# Autodesk Inventor assembly: benchtop-mesoSPIM-V2-1
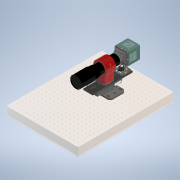
[picture p0: Inventor's stored thumbnail of the model, 180x180]
Saved by Autodesk Inventor 2021 (Build 250183000, 183)
## iProperties
Created: 2020-09-21
Part Number: benchtop-mesoSPIM-V2-1
Document SubType Name: Assembly
Designer: voigt
Author: voigt
## Documents named in this file (73)
- C:\Users\Public\mesoSPIM_design_benchtop\mesoSPIM\benchtop-mesoSPIM.iam
- C:\Users\Public\mesoSPIM_design_benchtop\library\Thorlabs\breadboards\PBG52522-Step.iam
- C:\Users\Public\mesoSPIM_design_benchtop\library\Thorlabs\accessoires\AV6_M.ipt
- C:\Users\Public\mesoSPIM_design_benchtop\library\Thorlabs\extrusions\XE25L375_M.ipt
- C:\Users\Public\mesoSPIM_design_benchtop\library\Thorlabs\extrusions\RM1S.ipt
- C:\Users\Public\mesoSPIM_design_benchtop\library\Thorlabs\extrusions\RM1G.ipt
- C:\Users\Public\mesoSPIM_design_benchtop\library\Thorlabs\extrusions\XE25L525_M.ipt
- C:\Users\Public\mesoSPIM_design_benchtop\library\Thorlabs\extrusions\XE25L350_M.ipt
- C:\Users\Public\mesoSPIM_design_benchtop\library\Thorlabs\accessoires\BBH1.ipt
- C:\Users\Public\mesoSPIM_design_benchtop\mesoSPIM\covers\Front_Cover_V1.ipt
- C:\Users\Public\mesoSPIM_design_benchtop\library\ASI\LS100_Vertical_Assembly.ipt
- C:\Users\Public\mesoSPIM_design_benchtop\library\ASI\ASI_mesoSPIM_Bridge.ipt
- C:\Users\Public\mesoSPIM_design_benchtop\library\ASI\LS-50HE ASSEMBLY (Centered Travel).ipt
- C:\Users\Public\mesoSPIM_design_benchtop\library\ASI\VTS-2112 DOVE RACK ASSEMBLY - (#DV6010 and #DV6020)_DV6010 ASSEMBLY with CDZ-SLIDE C.iam
- C:\Users\Public\mesoSPIM_design_benchtop\library\ASI\LS-50 LE ASSEMBLY_HOME.iam
- C:\Users\Public\mesoSPIM_design_benchtop\library\ASI\C60-3060-CMR-1011 - C-MOUNT TO LS50 SLIDE ADAPTER.ipt
- C:\Users\Public\mesoSPIM_design_benchtop\library\ASI\C60-3060-CMR - 3060 C-MOUNT ROTATING ASSEMBLY_C60-3060-CMR-Mo-ER20.iam
- C:\Users\Public\mesoSPIM_design_benchtop\library\ASI\LS-5012 - LS-BREADBOARD ADAPTER PLATE.ipt
- C:\Users\Public\mesoSPIM_design_benchtop\library\Thorlabs\rails\XT66SD.ipt
- C:\Users\Public\mesoSPIM_design_benchtop\library\Edmund_Optics\telecentric_objectives\62902_0_9x_F-Mount_PlatinumTL_Telecentric_lens.ipt
- C:\Users\Public\mesoSPIM_design_benchtop\library\Photometrics\Iris15_Volume_Correct.ipt
- C:\Users\Public\mesoSPIM_design_benchtop\library\Thorlabs\rails\XT66P2_M_single.ipt
- C:\Users\Public\mesoSPIM_design_benchtop\library\Thorlabs\posts\12_7_mm_posts\TR30.ipt
- C:\Users\Public\mesoSPIM_design_benchtop\library\Thorlabs\posts\post_mounts\PH20_M.ipt
- C:\Users\Public\mesoSPIM_design_benchtop\mesoSPIM\covers\Side_Cover_V1.ipt
- C:\Users\Public\mesoSPIM_design_benchtop\mesoSPIM\covers\Top_Cover_V1.ipt
- C:\Users\Public\mesoSPIM_design_benchtop\library\Thorlabs\extrusions\XE25H.ipt
- C:\Users\Public\mesoSPIM_design_benchtop\library\Thorlabs\posts\post_mounts\PH150_M.ipt
- C:\Users\Public\mesoSPIM_design_benchtop\library\Thorlabs\30mm_cage_system\cage_plates\CP33_M.ipt
- C:\Users\Public\mesoSPIM_design_benchtop\library\Thorlabs\posts\12_7_mm_posts\TR100M.ipt
- C:\Users\Public\mesoSPIM_design_benchtop\library\Thorlabs\30mm_cage_system\cage_rods\ER8_CageRod.ipt
- C:\Users\Public\mesoSPIM_design_benchtop\library\Thorlabs\optics\AC254-060-A-ML.ipt
- C:\Users\Public\mesoSPIM_design_benchtop\library\Thorlabs\accessoires\SM1FCA-APC-Fiberadapter.ipt
- C:\Users\Public\mesoSPIM_design_benchtop\library\Thorlabs\posts\post_mounts\PH40_M.ipt
- C:\Users\Public\mesoSPIM_design_benchtop\library\Thorlabs\posts\12_7_mm_posts\TR40M.ipt
- C:\Users\Public\mesoSPIM_design_benchtop\library\Thorlabs\30mm_cage_system\optics_mounts\KCB1E_M.ipt
- C:\Users\Public\mesoSPIM_design_benchtop\library\Thorlabs\optics\BBE1-E02-Step.ipt
- C:\Users\Public\mesoSPIM_design_benchtop\library\Thorlabs\optics\AC254-100-A-ML.ipt
- C:\Users\Public\mesoSPIM_design_benchtop\library\Optotune\EL-16-40\EL-16-40-TC-C (133-193-03-R0-01).iam
- C:\Users\Public\mesoSPIM_design_benchtop\library\Thorlabs\30mm_cage_system\SM1_tubes\SM1L10.ipt
- C:\Users\Public\mesoSPIM_design_benchtop\library\Thorlabs\accessoires\SM1A9.ipt
- C:\Users\Public\mesoSPIM_design_benchtop\library\Thorlabs\accessoires\SM1T2.ipt
- C:\Users\Public\mesoSPIM_design_benchtop\library\Thorlabs\accessoires\SM1NT.ipt
- C:\Users\Public\mesoSPIM_design_benchtop\library\Thorlabs\stages\XRN-B1_M-Micrometer-Baseplate.ipt
- C:\Users\Public\mesoSPIM_design_benchtop\library\Thorlabs\posts\post_mounts\PH75_M-Step.ipt
- C:\Users\Public\mesoSPIM_design_benchtop\library\Thorlabs\stages\XLN25P_M.ipt
- C:\Users\Public\mesoSPIM_design_benchtop\library\Thorlabs\stages\XRN25P_M.ipt
- C:\Users\Public\mesoSPIM_design_benchtop\library\Thorlabs\accessoires\AB90H.ipt
- C:\Users\Public\mesoSPIM_design_benchtop\library\Thorlabs\posts\12_7_mm_posts\TR75M.ipt
- C:\Users\Public\mesoSPIM_design_benchtop\library\Thorlabs\30mm_cage_system\cage_rods\ER0.5_CageRod.ipt
- C:\Users\Public\mesoSPIM_design_benchtop\library\Thorlabs\30mm_cage_system\cage_plates\CP30.ipt
- C:\Users\Public\mesoSPIM_design_benchtop\library\Thorlabs\30mm_cage_system\SM1_tubes\SM1L20.ipt
- C:\Users\Public\mesoSPIM_design_benchtop\library\Thorlabs\30mm_cage_system\SM1_tubes\SM1CPL.ipt
- C:\Users\Public\mesoSPIM_design_benchtop\library\Thorlabs\accessoires\BA1S_M.ipt
- C:\Users\Public\mesoSPIM_design_benchtop\library\Thorlabs\accessoires\MFF101_M_FlipMirror_SinglePart.ipt
- C:\Users\Public\mesoSPIM_design_benchtop\library\Thorlabs\optics\BB1-E02.ipt
- C:\Users\Public\mesoSPIM_design_benchtop\library\Thorlabs\60mm_cage_system\LCP03_M_modified_for_GVS411.ipt
- C:\Users\Public\mesoSPIM_design_benchtop\library\Thorlabs\galvos\GVS411-galvo-bracket-modified.ipt
- C:\Users\Public\mesoSPIM_design_benchtop\library\Thorlabs\galvos\GVS411_M.ipt
- C:\Users\Public\mesoSPIM_design_benchtop\mesoSPIM\excitation_path\components\60mm-blank-cageplate-LCP03M-Nikon-MOD.ipt
- C:\Users\Public\mesoSPIM_design_benchtop\library\Thorlabs\other\F-Mount-AdapterSM2NFM-Step.ipt
- C:\Users\Public\mesoSPIM_design_benchtop\library\Nikon\50mm_1_4G_body_disassembled.ipt
- C:\Users\Public\mesoSPIM_design_benchtop\library\Thorlabs\30mm_cage_system\cage_rods\ER4_CageRod.ipt
- C:\Users\Public\mesoSPIM_design_benchtop\mesoSPIM\sample_handling\Cuvette-Sampleholder\Cuvette-Sampleholder-with-base.iam
- C:\Users\Public\mesoSPIM_design_benchtop\library\Thorlabs\60mm_cage_system\LCFW5-wheel.ipt
- C:\Users\Public\mesoSPIM_design_benchtop\library\Robotis\MX-28T_R.ipt
- C:\Users\Public\mesoSPIM_design_benchtop\library\Robotis\FR07-S101.ipt
- C:\Users\nvladi\Documents\Inventor\mesoSPIM_design_benchtop_V2\library\Thorlabs\30mm_cage_system\cage_rods\ER_CageRod.ipt
- C:\Users\Public\mesoSPIM_design_benchtop\library\Lensation\T25M-12-155I.ipt
- C:\Users\Public\mesoSPIM_design_benchtop\mesoSPIM\detection_path\components\Lensagon1.2x-XT66P2M(ThorlabsRailCarriage).ipt
- C:\Users\Public\mesoSPIM_design_benchtop\library\Mouse_Brain\mousebrain2.ipt
- C:\Users\Public\mesoSPIM_design_benchtop\mesoSPIM\immersion_cuvette_mounts\ImmersionCuvetteAssembly.iam
- C:\Users\Public\mesoSPIM_design_benchtop\mesoSPIM\sample_handling\IDISCO-Sampleholder\Clamp-assembly.iam
## Components (172 placed, 71 different names)
1. AV6_M:4 — Mate:6, Mate:7
2. AV6_M:3 — Mate:8, Mate:9
3. AV6_M:2 — Mate:12, Mate:13
4. AV6_M:1 — Mate:10, Mate:11
5. PBG52522-Step:1 [sub-assembly] — Flush:1, Flush:2, Mate:5, Mate:6, Mate:7, Mate:8, Mate:9, Mate:10, Mate:11, Mate:12, Mate:13, Mate:14, Mate:15, Angle:1, Mate:16, Mate:17, Angle:2, Mate:18, Mate:19, Angle:3, Mate:20, Mate:21, Angle:4, Mate:32, Mate:48, Mate:49, Mate:50, Angle:5, Mate:51, Angle:6, Mate:72, Mate:107, Angle:15, Mate:109, Mate:110, Angle:16, Flush:45, Mate:139, Mate:140, Angle:18, Mate:141, Mate:142, Angle:19, Flush:49, Angle:20, Mate:191, Mate:192, Angle:23, Angle:24, Mate:196, Mate:197, Mate:198, Angle:25, Mate:199, Mate:200, Angle:26, Mate:238, Mate:239, Angle:28, Angle:30, Mate:243, Mate:324, Tangent:1, Mate:325, Mate:331, Angle:44, Mate:382, Angle:46, Tangent:2, Mate:385, Angle:47
6. LS100_Vertical_Assembly:1 — Mate:48, Mate:50, Angle:5, Mate:52, Mate:53
7. LS100_Vertical_Assembly:2 — Mate:49, Mate:51, Angle:6, Mate:54
8. ASI_mesoSPIM_Bridge:1 — Mate:52, Mate:53, Mate:54, Mate:55, Flush:36
9. LS-50HE ASSEMBLY (Centered Travel):1 — Mate:55, Flush:36, Mate:56, Mate:57, Angle:7, Mate:58, Mate:59, Angle:8
10. VTS-2112 DOVE RACK ASSEMBLY - (#DV6010 and #DV6020)_DV6010 ASSEMBLY with CDZ-SLIDE C:1 [sub-assembly] — Mate:57, Angle:7, Mate:58, Mate:59, Mate:60, Mate:61, Mate:62
11. LS-50 LE ASSEMBLY_HOME:1 [sub-assembly] — Mate:60, Mate:61, Mate:62, Angle:8, Mate:63, Mate:64, Mate:65
12. C60-3060-CMR-1011 - C-MOUNT TO LS50 SLIDE ADAPTER:1 — Mate:63, Mate:64, Mate:65, Mate:66, Mate:67
13. C60-3060-CMR - 3060 C-MOUNT ROTATING ASSEMBLY_C60-3060-CMR-Mo-ER20:1 [sub-assembly] — Mate:66, Mate:67, Mate:367, VerticalPos
14. LS-5012 - LS-BREADBOARD ADAPTER PLATE:1 — Mate:70, Angle:9, Mate:72, Mate:77
15. LS-50 LE ASSEMBLY_HOME:2 [sub-assembly] — Mate:70, Angle:9, Mate:73, Mate:74, Angle:10, Mate:77
16. XT66SD:1 — Mate:73, Mate:74, Angle:10, Mate:75, Mate:76, Angle:11, Mate:82, Mate:83, Mate:84, Mate:85
17. 62902_0_9x_F-Mount_PlatinumTL_Telecentric_lens:1 — Mate:78, Mate:81
18. Lensagon-T25M-12-155I:1 — Insert:3, Insert:7
19. Lensagon1.2x-XT66P2M(ThorlabsRailCarriage):1 — Mate:384, Flush:72, Flush:73, Insert:7
20. Iris15_Volume_Correct:1 — Angle:11, Mate:81, Insert:3, Insert:8
21. XT66P2_M_single:1 — Mate:82, Mate:83, Mate:96, Mate:97
22. XT66P2_M_single:2 — Mate:84, Mate:85, Mate:384, Flush:72, Flush:73
23. TR30:1 — Insert:8
24. PH20_M:1 — Mate:96, Mate:97
25. KCB1E_M:2 — Mate:184, Mate:185, Mate:186, Mate:187, Mate:188, Mate:190, Angle:21, Angle:36
26. BBE1-E02-Step:2 — Mate:189, Mate:190, Angle:21
27. CP33_M:2 — Mate:117, Mate:118, Mate:122
28. TR100M:1 — Mate:119
29. TR100M:2 — Mate:121, Mate:122
30. CP33_M:3 — Mate:124, Mate:129, Mate:131, Mate:133
31. CP33_M:4 — Mate:123, Flush:48, Mate:294
32. ER8_CageRod:1 — Mate:186, Mate:308
33. ER8_CageRod:2 — Mate:188, Mate:307
34. ER8_CageRod:3 — Mate:129, Mate:187, Mate:294
35. AC254-060-A-ML:1 — Mate:130, Mate:131
36. SM1FCA-APC-Fiberadapter:1 — Mate:132, Flush:48, Mate:133
37. PH150_M:1 — Mate:109, Mate:110, Angle:16, Mate:118, Mate:121
38. PH150_M:2 — Mate:107, Angle:15, Mate:119
39. LCP03_M_modified_for_GVS411:1 — Mate:337, Mate:338, Angle:39, Mate:349, Insert:2
40. GVS411-galvo-bracket-modified:1 — Mate:337, Mate:338, Mate:339, Angle:38, Angle:39, Mate:341
41. GVS411_M:1 — Mate:339, Angle:38, Mate:340, Mate:341, Mate:348
42. 60mm-blank-cageplate-LCP03M-Nikon-MOD:1 — Mate:344, Mate:345, Mate:347, Flush:66, Mate:350, Flush:67, Insert:1
43. F-Mount-AdapterSM2NFM-Step:1 — Mate:344, Mate:345, Mate:346
44. 50mm_1_4G_body_disassembled:1 — Mate:346, Mate:347, Mate:348
45. TR75M:2 — Mate:272
46. AB90H:1 — Mate:264, Mate:265, Flush:62
47. KCB1E_M:4 — Mate:254, Mate:255, Mate:258, Mate:259, Mate:265, Flush:62
48. BBE1-E02-Step:5 — Mate:258, Mate:259
49. XLN25P_M:1 — Mate:244, Mate:245, Mate:248, Mate:264
50. PH75_M-Step:2 — Mate:192, Angle:23, Mate:272
51. XRN-B1_M-Micrometer-Baseplate:1 — Mate:191, Angle:24, Mate:196, Mate:244, Mate:245
52. EL-16-40-TC-C (133-193-03-R0-01):1 [sub-assembly] — Mate:174, Mate:175, Mate:178, Mate:179
53. SM1L10:2 — Mate:176, Mate:177, Mate:181, Mate:182, Mate:183, Mate:185
54. SM1A9:1 — Mate:178, Mate:179, Mate:180
55. SM1T2:1 — Mate:180, Mate:181
56. SM1NT:1 — Mate:182, Mate:183
57. PH40_M:1 — Mate:139, Mate:140, Angle:18, Mate:148
58. PH40_M:2 — Mate:141, Mate:142, Angle:19, Mate:150
59. CP33_M:5 — Mate:147, Mate:148, Mate:153, Mate:154, Mate:155, Mate:156, Flush:53, Mate:159, Mate:160
60. CP33_M:6 — Mate:149, Mate:150, Mate:161, Mate:162
61. CP33_M:7 — Mate:151, Mate:157, Flush:54, Mate:169
62. ER8_CageRod:4 — Mate:156, Flush:51
63. ER8_CageRod:5 — Mate:155, Flush:50, Flush:51, Flush:52, Mate:157
64. ER8_CageRod:6 — Mate:154, Flush:52
65. ER8_CageRod:7 — Mate:153, Flush:50, Flush:53, Flush:54, Mate:164, Mate:165
66. TR40M:1 — Mate:159, Mate:160
67. TR40M:2 — Mate:161, Mate:162
68. KCB1E_M:1 — Mate:163, Mate:164, Mate:165, Mate:167, Mate:173, Mate:175, Mate:177
69. BBE1-E02-Step:1 — Mate:166, Mate:167, Angle:20
70. AC254-100-A-ML:1 — Mate:168, Mate:169
71. AC254-100-A-ML:2
72. ER4_CageRod:12 — Mate:349, Flush:66
73. ER4_CageRod:19 — Insert:1
74. ER4_CageRod:20 — Insert:2
75. ER4_CageRod:13 — Mate:350, Flush:67
76. LCP03_M_modified_for_GVS411:2 — Mate:352, Mate:353, Angle:41, Angle:43, Insert:10, Insert:11
77. GVS411-galvo-bracket-modified:2 — Mate:352, Mate:353, Angle:41, Mate:354, Angle:42, Mate:356
78. GVS411_M:2 — Mate:354, Angle:42, Mate:355, Mate:356, Mate:362
79. 60mm-blank-cageplate-LCP03M-Nikon-MOD:2 — Angle:43, Mate:358, Mate:359, Mate:361, Mate:365, Flush:70, Flush:71, Mate:366
80. F-Mount-AdapterSM2NFM-Step:2 — Mate:358, Mate:359, Mate:360
81. 50mm_1_4G_body_disassembled:2 — Mate:360, Mate:361, Mate:362
82. ER4_CageRod:14 — Mate:365, Flush:70
83. ER4_CageRod:16 — Flush:71, Mate:366
84. TR75M:4 — Mate:278
85. AB90H:2 — Mate:266, Mate:267, Flush:63
86. KCB1E_M:5 — Mate:256, Mate:257, Mate:261, Mate:267, Flush:63
87. BBE1-E02-Step:4 — Mate:260, Mate:261
88. XRN25P_M:1 — Mate:246, Mate:247, Mate:249, Mate:266
89. PH40_M:3 — Mate:197, Mate:198, Angle:25, Mate:205
90. PH40_M:4 — Mate:199, Mate:200, Angle:26, Mate:206
91. CP33_M:9 — Mate:201, Mate:205, Mate:207, Mate:208, Mate:211, Mate:212, Mate:213, Mate:214
92. CP33_M:10 — Mate:202, Mate:206, Mate:209, Mate:210, Flush:58
93. TR40M:3 — Mate:207, Mate:208
94. TR40M:4 — Mate:209, Mate:210
95. ER8_CageRod:8 — Mate:211, Flush:57, Flush:59
96. ER8_CageRod:9 — Mate:213, Flush:56, Flush:58, Mate:216, Mate:217, Mate:222
97. ER8_CageRod:10 — Mate:214, Flush:55, Flush:56, Flush:57
98. ER8_CageRod:11 — Mate:212, Flush:55
99. ER4_CageRod:21 — Insert:11
100. ER4_CageRod:22 — Insert:10
101. KCB1E_M:3 — Mate:215, Mate:216, Mate:217, Mate:219, Angle:27, Mate:227, Mate:228, Mate:229, Mate:231
102. BBE1-E02-Step:3 — Mate:218, Mate:219, Angle:27
103. CP33_M:11 — Mate:220, Flush:59, Mate:224
104. CP33_M:12 — Mate:221, Mate:222, Mate:226
105. AC254-100-A-ML:3 — Mate:223, Mate:224
106. AC254-100-A-ML:4 — Mate:225, Mate:226, Mate:227
107. SM1L10:3 — Mate:228, Mate:229, Mate:230, Mate:236, Mate:237, Mate:292
108. EL-16-40-TC-C (133-193-03-R0-01):2 [sub-assembly] — Mate:230, Mate:231, Mate:232, Mate:233
109. SM1A9:3 — Mate:232, Mate:233, Mate:234, Mate:235
110. SM1T2:2 — Mate:234, Mate:235
111. SM1NT:2 — Mate:236, Mate:237
112. XRN-B1_M-Micrometer-Baseplate:2 — Mate:238, Angle:30, Mate:243, Mate:246, Mate:247
113. PH75_M-Step:3 — Mate:239, Angle:28, Mate:278
114. CP33_M:13 — Mate:299, Mate:301, Mate:303, Mate:305, Mate:317
115. KCB1E_M:6 — Mate:292, Mate:296, Angle:32, Angle:35, Mate:300, Mate:302, Mate:314
116. KCB1E_M:7 — Mate:297, Angle:33, Angle:34, Mate:298, Angle:35, Mate:304, Mate:306, Mate:311, Mate:312, Mate:313, Mate:317, Mate:319, Mate:320
117. BBE1-E02-Step:6 — Mate:295, Mate:296, Angle:32
118. BBE1-E02-Step:7 — Mate:297, Angle:33, Angle:34, Mate:298
119. ER0.5_CageRod:1 — Mate:299, Mate:300, Mate:314
120. ER0.5_CageRod:2 — Mate:301, Mate:302
121. ER0.5_CageRod:3 — Mate:303, Mate:304, Mate:313
122. ER0.5_CageRod:4 — Mate:305, Mate:306
123. CP30:1 — Mate:307, Mate:308, Mate:309, Mate:310
124. SM1L20:1 — Mate:309, Mate:310, Mate:316
125. SM1L20:2 — Mate:311, Mate:312, Mate:316, Mate:318
126. SM1CPL:1 — Mate:318
127. TR100M:3 — Mate:319, Mate:320, Mate:321
128. PH150_M:3 — Mate:321, Mate:322, Mate:323
129. BA1S_M:1 — Mate:322, Mate:323, Mate:324, Tangent:1
130. BA1S_M:2 — Mate:325, Mate:326, Mate:327
131. PH75_M-Step:6 — Mate:326, Mate:327, Mate:328
132. TR75M:5 — Mate:328, Mate:329, Mate:330
133. MFF101_M_FlipMirror_SinglePart:1 — Mate:329, Mate:330, Angle:36, Mate:331, Mate:332, Mate:333
134. BB1-E02:1 — Mate:332, Mate:333
135. mousebrain2:1
136. TR40M:5 — Mate:367, VerticalPos, Mate:369, Mate:370, Insert:9
137. Clamp-assembly:1 [sub-assembly] — Insert:9, Angle:47
138. Cuvette-Sampleholder-with-base:1 [sub-assembly] — Mate:369, Mate:370, Angle:44
139. LCFW5-wheel:1 — Mate:371, Mate:372, Mate:373, Mate:383
140. MX-28T_R:1 — Mate:373, Mate:374, Mate:375, Mate:376, Mate:383
141. FR07-S101:1 — Mate:374, Mate:375, Mate:376, Mate:377, Mate:378
142. TR30:2 — Mate:377, Mate:378, Mate:379
143. PH20_M:2 — Mate:379, Mate:381, Angle:45
144. BA1S_M:3 — Mate:381, Mate:382, Angle:45, Angle:46, Tangent:2
145. ImmersionCuvetteAssembly:1 [sub-assembly] — Mate:385
146. XE25H:1 — Mate:103, Angle:14, Mate:104, Flush:43
147. XE25H:2 — Mate:105, Mate:106, Flush:44
148. XE25L525_M:1 — Mate:29, Flush:17, Flush:18, Mate:101, Flush:40, Flush:42
149. XE25L525_M:2 — Mate:28, Flush:15, Flush:16, Mate:100, Flush:38
150. XE25L375_M:5 — Mate:27, Flush:13, Flush:14, Flush:19, Mate:30, Flush:20, Mate:103, Flush:43, Mate:105, Flush:44
151. XE25L375_M:6 — Mate:26, Flush:11, Flush:12, Flush:41
152. RM1G:1 — Mate:22, Flush:3, Flush:4, Mate:28, Flush:15, Flush:16
153. RM1G:2 — Mate:24, Flush:7, Flush:8, Mate:26, Flush:11, Flush:12, Mate:29, Flush:17, Flush:18
154. RM1G:3 — Mate:25, Flush:9, Flush:10, Mate:27, Flush:13, Flush:14, Mate:104
155. RM1G:4 — Mate:23, Flush:5, Flush:6, Mate:102, Mate:106
156. XE25L375_M:1 — Mate:14, Mate:15, Angle:1, Mate:22, Flush:3, Flush:4, Flush:37
157. XE25L375_M:2 — Mate:16, Mate:17, Angle:2, Mate:24, Flush:7, Flush:8, Flush:39
158. XE25L375_M:3 — Mate:18, Mate:19, Angle:3, Mate:25, Flush:9, Flush:10
159. XE25L375_M:4 — Mate:20, Mate:21, Angle:4, Mate:23, Flush:5, Flush:6, Flush:21, Mate:31
160. Front_Cover_V1:1 — Mate:41, Mate:42, Mate:43
161. BBH1:1 — Mate:39, Flush:35, Mate:40
162. RM1S:1 — Mate:33, Flush:22, Flush:23
163. RM1S:2 — Mate:34, Flush:24, Flush:25, Flush:33, Flush:34, Mate:38
164. RM1S:3 — Flush:28, Mate:36, Flush:29, Flush:30, Mate:37, Flush:31, Flush:32
165. RM1S:4 — Mate:35, Flush:26, Flush:27
166. XE25L375_M:7 — Flush:19, Mate:30, Flush:20, Mate:34, Flush:24, Flush:25, Flush:28, Mate:36, Flush:29, Flush:30, Mate:43, Angle:14
167. XE25L375_M:8 — Flush:21, Mate:31, Mate:32, Mate:33, Flush:22, Flush:23, Mate:35, Flush:26, Flush:27, Mate:39, Flush:35
168. XE25L350_M:1 — Mate:37, Flush:31, Flush:32, Mate:41, Mate:42
169. XE25L350_M:2 — Flush:33, Flush:34, Mate:38
170. Side_Cover_V1:1 — Mate:100, Flush:37, Flush:38
171. Side_Cover_V1:2 — Mate:101, Flush:39, Flush:40
172. Top_Cover_V1:1 — Mate:102, Flush:41, Flush:42
## Relationships (418: Mate 302, Flush 67, Angle 39, Insert 8, Tangent 2)
- Flush:1 (135 mm): PBG52522-Step:1
- Flush:2 (225 mm): PBG52522-Step:1
- Mate:5 (-100 mm): PBG52522-Step:1
- Mate:6: AV6_M:4 ↔ PBG52522-Step:1
- Mate:7: AV6_M:4 ↔ PBG52522-Step:1
- Mate:8: AV6_M:3 ↔ PBG52522-Step:1
- Mate:9: AV6_M:3 ↔ PBG52522-Step:1
- Mate:10: AV6_M:1 ↔ PBG52522-Step:1
- Mate:11: AV6_M:1 ↔ PBG52522-Step:1
- Mate:12: AV6_M:2 ↔ PBG52522-Step:1
- Mate:13: AV6_M:2 ↔ PBG52522-Step:1
- Mate:14: PBG52522-Step:1 ↔ XE25L375_M:1
- Mate:15: PBG52522-Step:1 ↔ XE25L375_M:1
- Angle:1 (0 deg): PBG52522-Step:1 ↔ XE25L375_M:1
- Mate:16: PBG52522-Step:1 ↔ XE25L375_M:2
- Mate:17: PBG52522-Step:1 ↔ XE25L375_M:2
- Angle:2 (0 deg): PBG52522-Step:1 ↔ XE25L375_M:2
- Mate:18: PBG52522-Step:1 ↔ XE25L375_M:3
- Mate:19: PBG52522-Step:1 ↔ XE25L375_M:3
- Angle:3 (0 deg): PBG52522-Step:1 ↔ XE25L375_M:3
- Mate:20: PBG52522-Step:1 ↔ XE25L375_M:4
- Mate:21: PBG52522-Step:1 ↔ XE25L375_M:4
- Angle:4 (0 deg): PBG52522-Step:1 ↔ XE25L375_M:4
- Mate:22: RM1G:1 ↔ XE25L375_M:1
- Flush:3: RM1G:1 ↔ XE25L375_M:1
- Flush:4: RM1G:1 ↔ XE25L375_M:1
- Mate:23: RM1G:4 ↔ XE25L375_M:4
- Flush:5: RM1G:4 ↔ XE25L375_M:4
- Flush:6: RM1G:4 ↔ XE25L375_M:4
- Mate:24: RM1G:2 ↔ XE25L375_M:2
- Flush:7: RM1G:2 ↔ XE25L375_M:2
- Flush:8: RM1G:2 ↔ XE25L375_M:2
- Mate:25: RM1G:3 ↔ XE25L375_M:3
- Flush:9: RM1G:3 ↔ XE25L375_M:3
- Flush:10: RM1G:3 ↔ XE25L375_M:3
- Mate:26: XE25L375_M:6 ↔ RM1G:2
- Flush:11: XE25L375_M:6 ↔ RM1G:2
- Flush:12: XE25L375_M:6 ↔ RM1G:2
- Mate:27: XE25L375_M:5 ↔ RM1G:3
- Flush:13: XE25L375_M:5 ↔ RM1G:3
- Flush:14: XE25L375_M:5 ↔ RM1G:3
- Mate:28: XE25L525_M:2 ↔ RM1G:1
- Flush:15: XE25L525_M:2 ↔ RM1G:1
- Flush:16: XE25L525_M:2 ↔ RM1G:1
- Mate:29: XE25L525_M:1 ↔ RM1G:2
- Flush:17: XE25L525_M:1 ↔ RM1G:2
- Flush:18: XE25L525_M:1 ↔ RM1G:2
- Flush:19: XE25L375_M:5 ↔ XE25L375_M:7
- Mate:30: XE25L375_M:5 ↔ XE25L375_M:7
- Flush:20: XE25L375_M:5 ↔ XE25L375_M:7
- Flush:21 (-25 mm): XE25L375_M:4 ↔ XE25L375_M:8
- Mate:31: XE25L375_M:4 ↔ XE25L375_M:8
- Mate:32: PBG52522-Step:1 ↔ XE25L375_M:8
- Mate:33: RM1S:1 ↔ XE25L375_M:8
- Flush:22: RM1S:1 ↔ XE25L375_M:8
- Flush:23: RM1S:1 ↔ XE25L375_M:8
- Mate:34: RM1S:2 ↔ XE25L375_M:7
- Flush:24: RM1S:2 ↔ XE25L375_M:7
- Flush:25: RM1S:2 ↔ XE25L375_M:7
- Mate:35: RM1S:4 ↔ XE25L375_M:8
- Flush:26: RM1S:4 ↔ XE25L375_M:8
- Flush:27: RM1S:4 ↔ XE25L375_M:8
- Flush:28: RM1S:3 ↔ XE25L375_M:7
- Mate:36: RM1S:3 ↔ XE25L375_M:7
- Flush:29: RM1S:3 ↔ XE25L375_M:7
- Flush:30: RM1S:3 ↔ XE25L375_M:7
- Mate:37: RM1S:3 ↔ XE25L350_M:1
- Flush:31: RM1S:3 ↔ XE25L350_M:1
- Flush:32: RM1S:3 ↔ XE25L350_M:1
- Flush:33: RM1S:2 ↔ XE25L350_M:2
- Flush:34: RM1S:2 ↔ XE25L350_M:2
- Mate:38: RM1S:2 ↔ XE25L350_M:2
- Mate:39: BBH1:1 ↔ XE25L375_M:8
- Flush:35: BBH1:1 ↔ XE25L375_M:8
- Mate:40 (62.5 mm): BBH1:1
- Mate:41: Front_Cover_V1:1 ↔ XE25L350_M:1
- Mate:42 (-6 mm): Front_Cover_V1:1 ↔ XE25L350_M:1
- Mate:43 (-2 mm): Front_Cover_V1:1 ↔ XE25L375_M:7
- Mate:44
- Mate:45
- Mate:48: PBG52522-Step:1 ↔ LS100_Vertical_Assembly:1
- Mate:49: PBG52522-Step:1 ↔ LS100_Vertical_Assembly:2
- Mate:50: PBG52522-Step:1 ↔ LS100_Vertical_Assembly:1
- Angle:5 (0 deg): PBG52522-Step:1 ↔ LS100_Vertical_Assembly:1
- Mate:51: PBG52522-Step:1 ↔ LS100_Vertical_Assembly:2
- Angle:6 (0 deg): PBG52522-Step:1 ↔ LS100_Vertical_Assembly:2
- Mate:52: LS100_Vertical_Assembly:1 ↔ ASI_mesoSPIM_Bridge:1
- Mate:53: LS100_Vertical_Assembly:1 ↔ ASI_mesoSPIM_Bridge:1
- Mate:54: LS100_Vertical_Assembly:2 ↔ ASI_mesoSPIM_Bridge:1
- Mate:55: ASI_mesoSPIM_Bridge:1 ↔ LS-50HE ASSEMBLY (Centered Travel):1
- Flush:36: ASI_mesoSPIM_Bridge:1 ↔ LS-50HE ASSEMBLY (Centered Travel):1
- Mate:56 (12.5 mm): LS-50HE ASSEMBLY (Centered Travel):1
- Mate:57: LS-50HE ASSEMBLY (Centered Travel):1 ↔ VTS-2112 DOVE RACK ASSEMBLY - (#DV6010 and #DV6020)_DV6010 ASSEMBLY with CDZ-SLIDE C:1
- Angle:7 (0 deg): LS-50HE ASSEMBLY (Centered Travel):1 ↔ VTS-2112 DOVE RACK ASSEMBLY - (#DV6010 and #DV6020)_DV6010 ASSEMBLY with CDZ-SLIDE C:1
- Mate:58: LS-50HE ASSEMBLY (Centered Travel):1 ↔ VTS-2112 DOVE RACK ASSEMBLY - (#DV6010 and #DV6020)_DV6010 ASSEMBLY with CDZ-SLIDE C:1
- Mate:59: LS-50HE ASSEMBLY (Centered Travel):1 ↔ VTS-2112 DOVE RACK ASSEMBLY - (#DV6010 and #DV6020)_DV6010 ASSEMBLY with CDZ-SLIDE C:1
- Mate:60: VTS-2112 DOVE RACK ASSEMBLY - (#DV6010 and #DV6020)_DV6010 ASSEMBLY with CDZ-SLIDE C:1 ↔ LS-50 LE ASSEMBLY_HOME:1
- Mate:61: VTS-2112 DOVE RACK ASSEMBLY - (#DV6010 and #DV6020)_DV6010 ASSEMBLY with CDZ-SLIDE C:1 ↔ LS-50 LE ASSEMBLY_HOME:1
- Mate:62: VTS-2112 DOVE RACK ASSEMBLY - (#DV6010 and #DV6020)_DV6010 ASSEMBLY with CDZ-SLIDE C:1 ↔ LS-50 LE ASSEMBLY_HOME:1
- Angle:8 (0 deg): LS-50HE ASSEMBLY (Centered Travel):1 ↔ LS-50 LE ASSEMBLY_HOME:1
- Mate:63: LS-50 LE ASSEMBLY_HOME:1 ↔ C60-3060-CMR-1011 - C-MOUNT TO LS50 SLIDE ADAPTER:1
- Mate:64: LS-50 LE ASSEMBLY_HOME:1 ↔ C60-3060-CMR-1011 - C-MOUNT TO LS50 SLIDE ADAPTER:1
- Mate:65: LS-50 LE ASSEMBLY_HOME:1 ↔ C60-3060-CMR-1011 - C-MOUNT TO LS50 SLIDE ADAPTER:1
- Mate:66: C60-3060-CMR-1011 - C-MOUNT TO LS50 SLIDE ADAPTER:1 ↔ C60-3060-CMR - 3060 C-MOUNT ROTATING ASSEMBLY_C60-3060-CMR-Mo-ER20:1
- Mate:67: C60-3060-CMR-1011 - C-MOUNT TO LS50 SLIDE ADAPTER:1 ↔ C60-3060-CMR - 3060 C-MOUNT ROTATING ASSEMBLY_C60-3060-CMR-Mo-ER20:1
- Mate:70: LS-5012 - LS-BREADBOARD ADAPTER PLATE:1 ↔ LS-50 LE ASSEMBLY_HOME:2
- Angle:9 (0 deg): LS-5012 - LS-BREADBOARD ADAPTER PLATE:1 ↔ LS-50 LE ASSEMBLY_HOME:2
- Mate:72: PBG52522-Step:1 ↔ LS-5012 - LS-BREADBOARD ADAPTER PLATE:1
- Mate:73: LS-50 LE ASSEMBLY_HOME:2 ↔ XT66SD:1
- Mate:74: LS-50 LE ASSEMBLY_HOME:2 ↔ XT66SD:1
- Angle:10 (0 deg): LS-50 LE ASSEMBLY_HOME:2 ↔ XT66SD:1
- Mate:75: XT66SD:1
- Mate:76: XT66SD:1
- Mate:77: LS-5012 - LS-BREADBOARD ADAPTER PLATE:1 ↔ LS-50 LE ASSEMBLY_HOME:2
- Mate:78: 62902_0_9x_F-Mount_PlatinumTL_Telecentric_lens:1
- Angle:11 (0 deg): XT66SD:1 ↔ Iris15_Volume_Correct:1
- Mate:81: 62902_0_9x_F-Mount_PlatinumTL_Telecentric_lens:1 ↔ Iris15_Volume_Correct:1
- Mate:82: XT66SD:1 ↔ XT66P2_M_single:1
- Mate:83: XT66SD:1 ↔ XT66P2_M_single:1
- Mate:84: XT66SD:1 ↔ XT66P2_M_single:2
- Mate:85: XT66SD:1 ↔ XT66P2_M_single:2
- Mate:96: XT66P2_M_single:1 ↔ PH20_M:1
- Mate:97: XT66P2_M_single:1 ↔ PH20_M:1
- Mate:100: XE25L525_M:2 ↔ Side_Cover_V1:1
- Flush:37: XE25L375_M:1 ↔ Side_Cover_V1:1
- Flush:38: XE25L525_M:2 ↔ Side_Cover_V1:1
- Mate:101: XE25L525_M:1 ↔ Side_Cover_V1:2
- Flush:39: XE25L375_M:2 ↔ Side_Cover_V1:2
- Flush:40: XE25L525_M:1 ↔ Side_Cover_V1:2
- Mate:102: RM1G:4 ↔ Top_Cover_V1:1
- Flush:41: XE25L375_M:6 ↔ Top_Cover_V1:1
- Flush:42: XE25L525_M:1 ↔ Top_Cover_V1:1
- Mate:103: XE25H:1 ↔ XE25L375_M:5
- Angle:14 (0 deg): XE25H:1 ↔ XE25L375_M:7
- Mate:104: XE25H:1 ↔ RM1G:3
- Flush:43 (5.75 mm): XE25H:1 ↔ XE25L375_M:5
- Mate:105: XE25H:2 ↔ XE25L375_M:5
- Mate:106: XE25H:2 ↔ RM1G:4
- Flush:44 (5.75 mm): XE25H:2 ↔ XE25L375_M:5
- Mate:107: PBG52522-Step:1 ↔ PH150_M:2
- Angle:15 (0 deg): PBG52522-Step:1 ↔ PH150_M:2
- Mate:109: PBG52522-Step:1 ↔ PH150_M:1
- Mate:110: PBG52522-Step:1 ↔ PH150_M:1
- Angle:16 (0 deg): PBG52522-Step:1 ↔ PH150_M:1
- Flush:45 (215 mm): PBG52522-Step:1
- Flush:46 (-100 mm)
- Flush:47 (100 mm)
- Mate:111
- Mate:112
- Mate:113
- Mate:114
- Mate:117: CP33_M:2
- Mate:118: CP33_M:2 ↔ PH150_M:1
- Mate:119: TR100M:1 ↔ PH150_M:2
- Mate:121: TR100M:2 ↔ PH150_M:1
- Mate:122: CP33_M:2 ↔ TR100M:2
- Mate:123: CP33_M:4
- Mate:124: CP33_M:3
- Mate:129: CP33_M:3 ↔ ER8_CageRod:3
- Mate:130: AC254-060-A-ML:1
- Mate:131: CP33_M:3 ↔ AC254-060-A-ML:1
- Mate:132: SM1FCA-APC-Fiberadapter:1
- Flush:48 (-0.5 mm): CP33_M:4 ↔ SM1FCA-APC-Fiberadapter:1
- Mate:133 (50 mm): CP33_M:3 ↔ SM1FCA-APC-Fiberadapter:1
- Mate:139: PBG52522-Step:1 ↔ PH40_M:1
- Mate:140: PBG52522-Step:1 ↔ PH40_M:1
- Angle:18 (0 deg): PBG52522-Step:1 ↔ PH40_M:1
- Mate:141: PBG52522-Step:1 ↔ PH40_M:2
- Mate:142: PBG52522-Step:1 ↔ PH40_M:2
- Angle:19 (0 deg): PBG52522-Step:1 ↔ PH40_M:2
- Flush:49 (70 mm): PBG52522-Step:1
- Mate:143
- Mate:144
- Mate:145
- Mate:146
- Mate:147: CP33_M:5
- Mate:148: PH40_M:1 ↔ CP33_M:5
- Mate:149: CP33_M:6
- Mate:150: PH40_M:2 ↔ CP33_M:6
- Mate:151: CP33_M:7
- Mate:153: CP33_M:5 ↔ ER8_CageRod:7
- Mate:154: CP33_M:5 ↔ ER8_CageRod:6
- Mate:155: CP33_M:5 ↔ ER8_CageRod:5
- Mate:156: CP33_M:5 ↔ ER8_CageRod:4
- Flush:50: ER8_CageRod:5 ↔ ER8_CageRod:7
- Flush:51: ER8_CageRod:4 ↔ ER8_CageRod:5
- Flush:52: ER8_CageRod:5 ↔ ER8_CageRod:6
- Flush:53 (-39 mm): CP33_M:5 ↔ ER8_CageRod:7
- Mate:157: CP33_M:7 ↔ ER8_CageRod:5
- Mate:159: CP33_M:5 ↔ TR40M:1
- Mate:160: CP33_M:5 ↔ TR40M:1
- Mate:161: CP33_M:6 ↔ TR40M:2
- Mate:162: CP33_M:6 ↔ TR40M:2
- Flush:54: CP33_M:7 ↔ ER8_CageRod:7
- Mate:163: KCB1E_M:1
- Mate:164: ER8_CageRod:7 ↔ KCB1E_M:1
- Mate:165: ER8_CageRod:7 ↔ KCB1E_M:1
- Mate:166: BBE1-E02-Step:1
- Mate:167: KCB1E_M:1 ↔ BBE1-E02-Step:1
- Angle:20 (-90 deg): PBG52522-Step:1 ↔ BBE1-E02-Step:1
- Mate:168: AC254-100-A-ML:1
- Mate:169: CP33_M:7 ↔ AC254-100-A-ML:1
- Mate:173: KCB1E_M:1
- Mate:174: EL-16-40-TC-C (133-193-03-R0-01):1
- Mate:175 (35.6 mm): EL-16-40-TC-C (133-193-03-R0-01):1 ↔ KCB1E_M:1
- Mate:176: SM1L10:2
- Mate:177: SM1L10:2 ↔ KCB1E_M:1
- Mate:178: EL-16-40-TC-C (133-193-03-R0-01):1 ↔ SM1A9:1
- Mate:179: EL-16-40-TC-C (133-193-03-R0-01):1 ↔ SM1A9:1
- Mate:180: SM1A9:1 ↔ SM1T2:1
- Mate:181: SM1L10:2 ↔ SM1T2:1
- Mate:182: SM1L10:2 ↔ SM1NT:1
- Mate:183: SM1L10:2 ↔ SM1NT:1
- Mate:184: KCB1E_M:2
- Mate:185: KCB1E_M:2 ↔ SM1L10:2
- Mate:186: KCB1E_M:2 ↔ ER8_CageRod:1
- Mate:187: KCB1E_M:2 ↔ ER8_CageRod:3
- Mate:188: KCB1E_M:2 ↔ ER8_CageRod:2
- Mate:189: BBE1-E02-Step:2
- Mate:190: KCB1E_M:2 ↔ BBE1-E02-Step:2
- Angle:21 (0 deg): KCB1E_M:2 ↔ BBE1-E02-Step:2
- Mate:191: PBG52522-Step:1 ↔ XRN-B1_M-Micrometer-Baseplate:1
- Mate:192: PBG52522-Step:1 ↔ PH75_M-Step:2
- Angle:23 (0 deg): PBG52522-Step:1 ↔ PH75_M-Step:2
- Angle:24 (0 deg): PBG52522-Step:1 ↔ XRN-B1_M-Micrometer-Baseplate:1
- Mate:196: PBG52522-Step:1 ↔ XRN-B1_M-Micrometer-Baseplate:1
- Mate:197: PBG52522-Step:1 ↔ PH40_M:3
- Mate:198: PBG52522-Step:1 ↔ PH40_M:3
- Angle:25 (0 deg): PBG52522-Step:1 ↔ PH40_M:3
- Mate:199: PBG52522-Step:1 ↔ PH40_M:4
- Mate:200: PBG52522-Step:1 ↔ PH40_M:4
- Angle:26 (0 deg): PBG52522-Step:1 ↔ PH40_M:4
- Mate:201: CP33_M:9
- Mate:202: CP33_M:10
- Mate:205: PH40_M:3 ↔ CP33_M:9
- Mate:206: PH40_M:4 ↔ CP33_M:10
- Mate:207: CP33_M:9 ↔ TR40M:3
- Mate:208: CP33_M:9 ↔ TR40M:3
- Mate:209: CP33_M:10 ↔ TR40M:4
- Mate:210: CP33_M:10 ↔ TR40M:4
- Mate:211: CP33_M:9 ↔ ER8_CageRod:8
- Mate:212: CP33_M:9 ↔ ER8_CageRod:11
- Mate:213: CP33_M:9 ↔ ER8_CageRod:9
- Mate:214: CP33_M:9 ↔ ER8_CageRod:10
- Flush:55: ER8_CageRod:10 ↔ ER8_CageRod:11
- Flush:56: ER8_CageRod:9 ↔ ER8_CageRod:10
- Flush:57: ER8_CageRod:8 ↔ ER8_CageRod:10
- Flush:58 (-39 mm): CP33_M:10 ↔ ER8_CageRod:9
- Mate:215: KCB1E_M:3
- Mate:216: ER8_CageRod:9 ↔ KCB1E_M:3
- Mate:217: ER8_CageRod:9 ↔ KCB1E_M:3
- Mate:218: BBE1-E02-Step:3
- Mate:219: KCB1E_M:3 ↔ BBE1-E02-Step:3
- Angle:27 (0 deg): KCB1E_M:3 ↔ BBE1-E02-Step:3
- Mate:220: CP33_M:11
- Mate:221: CP33_M:12
- Mate:222: ER8_CageRod:9 ↔ CP33_M:12
- Flush:59: ER8_CageRod:8 ↔ CP33_M:11
- Mate:223: AC254-100-A-ML:3
- Mate:224: CP33_M:11 ↔ AC254-100-A-ML:3
- Mate:225: AC254-100-A-ML:4
- Mate:226: CP33_M:12 ↔ AC254-100-A-ML:4
- Mate:227 (0.5 mm): KCB1E_M:3 ↔ AC254-100-A-ML:4
- Mate:228: KCB1E_M:3 ↔ SM1L10:3
- Mate:229: KCB1E_M:3 ↔ SM1L10:3
- Mate:230: SM1L10:3 ↔ EL-16-40-TC-C (133-193-03-R0-01):2
- Mate:231 (35.6 mm): KCB1E_M:3 ↔ EL-16-40-TC-C (133-193-03-R0-01):2
- Mate:232: EL-16-40-TC-C (133-193-03-R0-01):2 ↔ SM1A9:3
- Mate:233: EL-16-40-TC-C (133-193-03-R0-01):2 ↔ SM1A9:3
- Mate:234: SM1A9:3 ↔ SM1T2:2
- Mate:235: SM1A9:3 ↔ SM1T2:2
- Mate:236: SM1L10:3 ↔ SM1NT:2
- Mate:237: SM1L10:3 ↔ SM1NT:2
- Mate:238: PBG52522-Step:1 ↔ XRN-B1_M-Micrometer-Baseplate:2
- Mate:239: PBG52522-Step:1 ↔ PH75_M-Step:3
- Angle:28 (0 deg): PBG52522-Step:1 ↔ PH75_M-Step:3
- Angle:30 (0 deg): PBG52522-Step:1 ↔ XRN-B1_M-Micrometer-Baseplate:2
- Mate:243: PBG52522-Step:1 ↔ XRN-B1_M-Micrometer-Baseplate:2
- Mate:244: XLN25P_M:1 ↔ XRN-B1_M-Micrometer-Baseplate:1
- Mate:245: XLN25P_M:1 ↔ XRN-B1_M-Micrometer-Baseplate:1
- Mate:246: XRN25P_M:1 ↔ XRN-B1_M-Micrometer-Baseplate:2
- Mate:247: XRN25P_M:1 ↔ XRN-B1_M-Micrometer-Baseplate:2
- Mate:248: XLN25P_M:1
- Mate:249: XRN25P_M:1
- Mate:250
- Mate:251
- Mate:252
- Mate:253
- Mate:254: KCB1E_M:4
- Mate:255: KCB1E_M:4
- Mate:256: KCB1E_M:5
- Mate:257: KCB1E_M:5
- Mate:258: KCB1E_M:4 ↔ BBE1-E02-Step:5
- Mate:259: KCB1E_M:4 ↔ BBE1-E02-Step:5
- Mate:260: BBE1-E02-Step:4
- Mate:261: KCB1E_M:5 ↔ BBE1-E02-Step:4
- Mate:262
- Mate:263
- Mate:264: AB90H:1 ↔ XLN25P_M:1
- Mate:265: AB90H:1 ↔ KCB1E_M:4
- Flush:62 (-8.1 mm): AB90H:1 ↔ KCB1E_M:4
- Mate:266: AB90H:2 ↔ XRN25P_M:1
- Mate:267: AB90H:2 ↔ KCB1E_M:5
- Flush:63 (8.1 mm): AB90H:2 ↔ KCB1E_M:5
- Mate:272: TR75M:2 ↔ PH75_M-Step:2
- Mate:278: TR75M:4 ↔ PH75_M-Step:3
- Mate:292: SM1L10:3 ↔ KCB1E_M:6
- Mate:294: CP33_M:4 ↔ ER8_CageRod:3
- Mate:295: BBE1-E02-Step:6
- Mate:296: KCB1E_M:6 ↔ BBE1-E02-Step:6
- Angle:32 (0 deg): KCB1E_M:6 ↔ BBE1-E02-Step:6
- Mate:297: KCB1E_M:7 ↔ BBE1-E02-Step:7
- Angle:33 (0 deg): KCB1E_M:7 ↔ BBE1-E02-Step:7
- Angle:34 (0 deg): KCB1E_M:7 ↔ BBE1-E02-Step:7
- Mate:298: KCB1E_M:7 ↔ BBE1-E02-Step:7
- Angle:35 (0 deg): KCB1E_M:6 ↔ KCB1E_M:7
- Mate:299: CP33_M:13 ↔ ER0.5_CageRod:1
- Mate:300: KCB1E_M:6 ↔ ER0.5_CageRod:1
- Mate:301: CP33_M:13 ↔ ER0.5_CageRod:2
- Mate:302: KCB1E_M:6 ↔ ER0.5_CageRod:2
- Mate:303: CP33_M:13 ↔ ER0.5_CageRod:3
- Mate:304: KCB1E_M:7 ↔ ER0.5_CageRod:3
- Mate:305: CP33_M:13 ↔ ER0.5_CageRod:4
- Mate:306: KCB1E_M:7 ↔ ER0.5_CageRod:4
- Mate:307: ER8_CageRod:2 ↔ CP30:1
- Mate:308: ER8_CageRod:1 ↔ CP30:1
- Mate:309: CP30:1 ↔ SM1L20:1
- Mate:310: CP30:1 ↔ SM1L20:1
- Mate:311: KCB1E_M:7 ↔ SM1L20:2
- Mate:312: KCB1E_M:7 ↔ SM1L20:2
- Mate:313: KCB1E_M:7 ↔ ER0.5_CageRod:3
- Mate:314: KCB1E_M:6 ↔ ER0.5_CageRod:1
- Mate:316: SM1L20:1 ↔ SM1L20:2
- Mate:317 (4 mm): CP33_M:13 ↔ KCB1E_M:7
- Mate:318: SM1L20:2 ↔ SM1CPL:1
- Mate:319: KCB1E_M:7 ↔ TR100M:3
- Mate:320: KCB1E_M:7 ↔ TR100M:3
- Mate:321: TR100M:3 ↔ PH150_M:3
- Mate:322: PH150_M:3 ↔ BA1S_M:1
- Mate:323: PH150_M:3 ↔ BA1S_M:1
- Mate:324: PBG52522-Step:1 ↔ BA1S_M:1
- Tangent:1: PBG52522-Step:1 ↔ BA1S_M:1
- Mate:325: PBG52522-Step:1 ↔ BA1S_M:2
- Mate:326: BA1S_M:2 ↔ PH75_M-Step:6
- Mate:327: BA1S_M:2 ↔ PH75_M-Step:6
- Mate:328: PH75_M-Step:6 ↔ TR75M:5
- Mate:329: TR75M:5 ↔ MFF101_M_FlipMirror_SinglePart:1
- Mate:330: TR75M:5 ↔ MFF101_M_FlipMirror_SinglePart:1
- Angle:36 (-135 deg): KCB1E_M:2 ↔ MFF101_M_FlipMirror_SinglePart:1
- Mate:331 (214 mm): PBG52522-Step:1 ↔ MFF101_M_FlipMirror_SinglePart:1
- Mate:332: MFF101_M_FlipMirror_SinglePart:1 ↔ BB1-E02:1
- Mate:333: MFF101_M_FlipMirror_SinglePart:1 ↔ BB1-E02:1
- Mate:337: LCP03_M_modified_for_GVS411:1 ↔ GVS411-galvo-bracket-modified:1
- Mate:338: LCP03_M_modified_for_GVS411:1 ↔ GVS411-galvo-bracket-modified:1
- Mate:339: GVS411-galvo-bracket-modified:1 ↔ GVS411_M:1
- Angle:38 (45 deg): GVS411-galvo-bracket-modified:1 ↔ GVS411_M:1
- Mate:340: GVS411_M:1
- Angle:39 (0 deg): LCP03_M_modified_for_GVS411:1 ↔ GVS411-galvo-bracket-modified:1
- Mate:341 (1 mm): GVS411-galvo-bracket-modified:1 ↔ GVS411_M:1
- Mate:344: 60mm-blank-cageplate-LCP03M-Nikon-MOD:1 ↔ F-Mount-AdapterSM2NFM-Step:1
- Mate:345: 60mm-blank-cageplate-LCP03M-Nikon-MOD:1 ↔ F-Mount-AdapterSM2NFM-Step:1
- Mate:346: F-Mount-AdapterSM2NFM-Step:1 ↔ 50mm_1_4G_body_disassembled:1
- Mate:347: 60mm-blank-cageplate-LCP03M-Nikon-MOD:1 ↔ 50mm_1_4G_body_disassembled:1
- Mate:348 (12 mm): GVS411_M:1 ↔ 50mm_1_4G_body_disassembled:1
- Mate:349: LCP03_M_modified_for_GVS411:1 ↔ ER4_CageRod:12
- Flush:66: 60mm-blank-cageplate-LCP03M-Nikon-MOD:1 ↔ ER4_CageRod:12
- Mate:350: 60mm-blank-cageplate-LCP03M-Nikon-MOD:1 ↔ ER4_CageRod:13
- Flush:67: 60mm-blank-cageplate-LCP03M-Nikon-MOD:1 ↔ ER4_CageRod:13
- Mate:352: LCP03_M_modified_for_GVS411:2 ↔ GVS411-galvo-bracket-modified:2
- Mate:353: LCP03_M_modified_for_GVS411:2 ↔ GVS411-galvo-bracket-modified:2
- Angle:41 (0 deg): LCP03_M_modified_for_GVS411:2 ↔ GVS411-galvo-bracket-modified:2
- Mate:354: GVS411-galvo-bracket-modified:2 ↔ GVS411_M:2
- Angle:42 (-45 deg): GVS411-galvo-bracket-modified:2 ↔ GVS411_M:2
- Mate:355: GVS411_M:2
- Mate:356 (1 mm): GVS411-galvo-bracket-modified:2 ↔ GVS411_M:2
- Angle:43 (0 deg): LCP03_M_modified_for_GVS411:2 ↔ 60mm-blank-cageplate-LCP03M-Nikon-MOD:2
- Mate:358: 60mm-blank-cageplate-LCP03M-Nikon-MOD:2 ↔ F-Mount-AdapterSM2NFM-Step:2
- Mate:359: 60mm-blank-cageplate-LCP03M-Nikon-MOD:2 ↔ F-Mount-AdapterSM2NFM-Step:2
- Mate:360: F-Mount-AdapterSM2NFM-Step:2 ↔ 50mm_1_4G_body_disassembled:2
- Mate:361: 60mm-blank-cageplate-LCP03M-Nikon-MOD:2 ↔ 50mm_1_4G_body_disassembled:2
- Mate:362 (12 mm): GVS411_M:2 ↔ 50mm_1_4G_body_disassembled:2
- Mate:365: 60mm-blank-cageplate-LCP03M-Nikon-MOD:2 ↔ ER4_CageRod:14
- Flush:70: 60mm-blank-cageplate-LCP03M-Nikon-MOD:2 ↔ ER4_CageRod:14
- Flush:71: 60mm-blank-cageplate-LCP03M-Nikon-MOD:2 ↔ ER4_CageRod:16
- Mate:366: 60mm-blank-cageplate-LCP03M-Nikon-MOD:2 ↔ ER4_CageRod:16
- Mate:367: C60-3060-CMR - 3060 C-MOUNT ROTATING ASSEMBLY_C60-3060-CMR-Mo-ER20:1 ↔ TR40M:5
- VerticalPos [Mate] (6 mm): C60-3060-CMR - 3060 C-MOUNT ROTATING ASSEMBLY_C60-3060-CMR-Mo-ER20:1 ↔ TR40M:5
- Mate:369: TR40M:5 ↔ Cuvette-Sampleholder-with-base:1
- Mate:370: TR40M:5 ↔ Cuvette-Sampleholder-with-base:1
- Angle:44 (0 deg): PBG52522-Step:1 ↔ Cuvette-Sampleholder-with-base:1
- Mate:371: LCFW5-wheel:1
- Mate:372: LCFW5-wheel:1
- Mate:373: LCFW5-wheel:1 ↔ MX-28T_R:1
- Mate:374: MX-28T_R:1 ↔ FR07-S101:1
- Mate:375: MX-28T_R:1 ↔ FR07-S101:1
- Mate:376: MX-28T_R:1 ↔ FR07-S101:1
- Mate:377: FR07-S101:1 ↔ TR30:2
- Mate:378: FR07-S101:1 ↔ TR30:2
- Mate:379: TR30:2 ↔ PH20_M:2
- Mate:381: PH20_M:2 ↔ BA1S_M:3
- Mate:382: PBG52522-Step:1 ↔ BA1S_M:3
- Mate:383 (4 mm): LCFW5-wheel:1 ↔ MX-28T_R:1
- Angle:45 (0 deg): PH20_M:2 ↔ BA1S_M:3
- Angle:46 (0 deg): PBG52522-Step:1 ↔ BA1S_M:3
- Tangent:2: PBG52522-Step:1 ↔ BA1S_M:3
- Insert:1 (-6 mm): 60mm-blank-cageplate-LCP03M-Nikon-MOD:1 ↔ ER4_CageRod:19
- Insert:2: LCP03_M_modified_for_GVS411:1 ↔ ER4_CageRod:20
- Insert:3: Lensagon-T25M-12-155I:1 ↔ Iris15_Volume_Correct:1
- Mate:384: Lensagon1.2x-XT66P2M(ThorlabsRailCarriage):1 ↔ XT66P2_M_single:2
- Flush:72: Lensagon1.2x-XT66P2M(ThorlabsRailCarriage):1 ↔ XT66P2_M_single:2
- Flush:73: Lensagon1.2x-XT66P2M(ThorlabsRailCarriage):1 ↔ XT66P2_M_single:2
- Mate:385: PBG52522-Step:1 ↔ ImmersionCuvetteAssembly:1
- Insert:7: Lensagon-T25M-12-155I:1 ↔ Lensagon1.2x-XT66P2M(ThorlabsRailCarriage):1
- Insert:8: Iris15_Volume_Correct:1 ↔ TR30:1
- Insert:9 (-5 mm): TR40M:5 ↔ Clamp-assembly:1
- Angle:47 (0 deg): PBG52522-Step:1 ↔ Clamp-assembly:1
- Insert:10: LCP03_M_modified_for_GVS411:2 ↔ ER4_CageRod:22
- Insert:11: LCP03_M_modified_for_GVS411:2 ↔ ER4_CageRod:21
